# Autodesk Inventor assembly: Anglerfish_lunchbox_m12large_flipped_v0
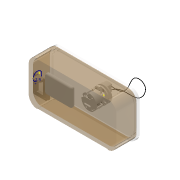
[picture p0: Inventor's stored thumbnail of the model, 180x180]
Saved by Autodesk Inventor 2022 (Build 260153000, 153)
## iProperties
Created: 2022-04-02
Part Number: Anglerfish_lunchbox_m12large_flipped_v0
Document SubType Name: Assembly
Designer: Prakash Lab
Author: Prakash Lab
## Documents named in this file (16)
- C:\Users\diederichbenedict\Dropbox\Dokumente\Promotion\PROJECTS\Matchboxscope\INVENTOR\RELEASE\Anglerfish\Workspace\Anglerfish_lunchbox_m12large_flipped_v0.iam
- C:\Users\diederichbenedict\Dropbox\Dokumente\Promotion\PROJECTS\Matchboxscope\INVENTOR\RELEASE\Anglerfish\Workspace\00_ESP3-CAM.iam
- C:\Users\diederichbenedict\Dropbox\Dokumente\Promotion\PROJECTS\Matchboxscope\INVENTOR\RELEASE\Anglerfish\Workspace\00_Powerbank.ipt
- C:\Users\diederichbenedict\Dropbox\Dokumente\Promotion\PROJECTS\Matchboxscope\INVENTOR\RELEASE\Anglerfish\Workspace\Matchboxscope_M12_Lensadapter_v0.ipt
- C:\Users\diederichbenedict\Dropbox\Dokumente\Promotion\PROJECTS\Matchboxscope\INVENTOR\RELEASE\Anglerfish\Workspace\00_CCTV_M12_VCM_large.ipt
- C:\Users\diederichbenedict\Dropbox\Dokumente\Promotion\PROJECTS\Matchboxscope\INVENTOR\RELEASE\Anglerfish\Workspace\Anglerfish_flipped_LidMoun.ipt
- C:\Users\diederichbenedict\Dropbox\Dokumente\Promotion\PROJECTS\Matchboxscope\INVENTOR\RELEASE\Anglerfish\Workspace\Anglerfish_flipped_Baselayer.ipt
- C:\Users\diederichbenedict\Dropbox\Dokumente\Promotion\PROJECTS\Matchboxscope\INVENTOR\RELEASE\Anglerfish\Workspace\Anglerfish_flipped_Electronicsmount.ipt
- C:\Users\diederichbenedict\Dropbox\Dokumente\Promotion\PROJECTS\Matchboxscope\INVENTOR\RELEASE\Anglerfish\Workspace\00_Magnet_8x3mm.ipt
- C:\Users\diederichbenedict\Dropbox\Dokumente\Promotion\PROJECTS\Matchboxscope\INVENTOR\RELEASE\Anglerfish\Workspace\DIN 912 - M3 x 0.5 x 12 x 10.75.ipt
- C:\Users\diederichbenedict\Dropbox\Dokumente\Promotion\PROJECTS\Matchboxscope\INVENTOR\RELEASE\Anglerfish\Workspace\00_Toslink.ipt
- C:\Users\diederichbenedict\Dropbox\Dokumente\Promotion\PROJECTS\Matchboxscope\INVENTOR\RELEASE\Anglerfish\Workspace\00_lunchbox_body.ipt
- C:\Users\diederichbenedict\Dropbox\Dokumente\Promotion\PROJECTS\Matchboxscope\INVENTOR\RELEASE\Anglerfish\Workspace\00_Lunchbox_cover.ipt
- C:\Users\diederichbenedict\Dropbox\Dokumente\Promotion\PROJECTS\Matchboxscope\INVENTOR\RELEASE\Anglerfish\Workspace\Matchboxscope_sample_universal_toslink.ipt
- C:\Users\diederichbenedict\Dropbox\Dokumente\Promotion\PROJECTS\Matchboxscope\INVENTOR\RELEASE\Anglerfish\Workspace\Anglerfish_coverslipclamp_top.ipt
- C:\Users\diederichbenedict\Dropbox\Dokumente\Promotion\PROJECTS\Matchboxscope\INVENTOR\RELEASE\Anglerfish\Workspace\Anglerfish_coverslipclamp_levelarm.ipt
## Components (27 placed, 15 different names)
1. 00_Powerbank:1
2. 00_ESP3-CAM:1 [sub-assembly] — Passend:23, Passend:24, Winkel:9, Winkel:11
3. 00_CCTV_M12_VCM_large:1 — Passend:30, Fluchtend:3, Einfügen:11
4. Matchboxscope_M12_Lensadapter_v0:1 — Einfügen:11
5. Anglerfish_flipped_Electronicsmount:1 — Einfügen:2, Winkel:11, Passend:30
6. Anglerfish_flipped_Baselayer:1 — Passend:23, Passend:24, Winkel:9, Einfügen:2, Winkel:10, Fluchtend:3, Einfügen:8, Einfügen:9, Einfügen:10, Einfügen:12, Einfügen:13, Einfügen:14, Einfügen:15, Einfügen:16, Einfügen:17, Einfügen:18
7. 00_Magnet_8x3mm:2 — Einfügen:21
8. 00_Magnet_8x3mm:3 — Einfügen:9
9. 00_Magnet_8x3mm:4 — Einfügen:20
10. 00_Magnet_8x3mm:5 — Einfügen:8
11. 00_Magnet_8x3mm:6 — Einfügen:10
12. DIN 912 - replaced by DIN EN ISO 4762 M3 x 12:1 — Einfügen:14
13. DIN 912 - replaced by DIN EN ISO 4762 M3 x 12:2 — Einfügen:17
14. DIN 912 - replaced by DIN EN ISO 4762 M3 x 12:4 — Einfügen:15
15. DIN 912 - replaced by DIN EN ISO 4762 M3 x 12:5 — Einfügen:12
16. DIN 912 - replaced by DIN EN ISO 4762 M3 x 12:6 — Einfügen:16
17. DIN 912 - replaced by DIN EN ISO 4762 M3 x 12:7 — Einfügen:13
18. 00_Toslink:1 — Einfügen:23
19. 00_lunchbox_body:1 — Fluchtend:4, Winkel:14, Fluchtend:33, Fluchtend:34, Passend:31
20. 00_Lunchbox_cover:1 — Fluchtend:33, Fluchtend:34, Passend:31, Fluchtend:35
21. Anglerfish_flipped_LidMoun:1 — Einfügen:18, Fluchtend:35, Einfügen:19, Einfügen:20, Einfügen:21, Einfügen:22
22. 00_Magnet_8x3mm:7 — Einfügen:19
23. Matchboxscope_M12_Lensadapter_v0:2 — Einfügen:24
24. Matchboxscope_sample_universal_toslink:2 — Einfügen:22, Einfügen:23, Einfügen:24
25. 00_Powerbank:2
26. Anglerfish_coverslipclamp_top:1 — Fluchtend:36, Fluchtend:37
27. Anglerfish_coverslipclamp_levelarm:1 — Fluchtend:36, Fluchtend:37
## Relationships (33: Insert 18, Flush 7, Mate 4, Angle 4)
- Passend:23 [Mate]: 00_ESP3-CAM:1 ↔ Anglerfish_flipped_Baselayer:1
- Passend:24 [Mate]: 00_ESP3-CAM:1 ↔ Anglerfish_flipped_Baselayer:1
- Winkel:9 [Angle] (180 deg): 00_ESP3-CAM:1 ↔ Anglerfish_flipped_Baselayer:1
- Einfügen:2 [Insert]: Anglerfish_flipped_Electronicsmount:1 ↔ Anglerfish_flipped_Baselayer:1
- Winkel:10 [Angle] (180 deg): Anglerfish_flipped_Baselayer:1
- Winkel:11 [Angle] (180 deg): 00_ESP3-CAM:1 ↔ Anglerfish_flipped_Electronicsmount:1
- Passend:30 [Mate]: 00_CCTV_M12_VCM_large:1 ↔ Anglerfish_flipped_Electronicsmount:1
- Fluchtend:3 [Flush]: 00_CCTV_M12_VCM_large:1 ↔ Anglerfish_flipped_Baselayer:1
- Einfügen:8 [Insert]: Anglerfish_flipped_Baselayer:1 ↔ 00_Magnet_8x3mm:5
- Einfügen:9 [Insert]: Anglerfish_flipped_Baselayer:1 ↔ 00_Magnet_8x3mm:3
- Einfügen:10 [Insert]: Anglerfish_flipped_Baselayer:1 ↔ 00_Magnet_8x3mm:6
- Einfügen:11 [Insert]: 00_CCTV_M12_VCM_large:1 ↔ Matchboxscope_M12_Lensadapter_v0:1
- Einfügen:12 [Insert]: Anglerfish_flipped_Baselayer:1 ↔ DIN 912 - replaced by DIN EN ISO 4762 M3 x 12:5
- Einfügen:13 [Insert]: Anglerfish_flipped_Baselayer:1 ↔ DIN 912 - replaced by DIN EN ISO 4762 M3 x 12:7
- Einfügen:14 [Insert]: Anglerfish_flipped_Baselayer:1 ↔ DIN 912 - replaced by DIN EN ISO 4762 M3 x 12:1
- Einfügen:15 [Insert]: Anglerfish_flipped_Baselayer:1 ↔ DIN 912 - replaced by DIN EN ISO 4762 M3 x 12:4
- Einfügen:16 [Insert]: Anglerfish_flipped_Baselayer:1 ↔ DIN 912 - replaced by DIN EN ISO 4762 M3 x 12:6
- Einfügen:17 [Insert]: Anglerfish_flipped_Baselayer:1 ↔ DIN 912 - replaced by DIN EN ISO 4762 M3 x 12:2
- Fluchtend:4 [Flush]: 00_lunchbox_body:1
- Winkel:14 [Angle] (180 deg): 00_lunchbox_body:1
- Fluchtend:33 [Flush]: 00_lunchbox_body:1 ↔ 00_Lunchbox_cover:1
- Fluchtend:34 [Flush]: 00_lunchbox_body:1 ↔ 00_Lunchbox_cover:1
- Passend:31 [Mate]: 00_lunchbox_body:1 ↔ 00_Lunchbox_cover:1
- Einfügen:18 [Insert] (-20 mm): Anglerfish_flipped_Baselayer:1 ↔ Anglerfish_flipped_LidMoun:1
- Fluchtend:35 [Flush] (-5 mm): 00_Lunchbox_cover:1 ↔ Anglerfish_flipped_LidMoun:1
- Einfügen:19 [Insert]: Anglerfish_flipped_LidMoun:1 ↔ 00_Magnet_8x3mm:7
- Einfügen:20 [Insert]: 00_Magnet_8x3mm:4 ↔ Anglerfish_flipped_LidMoun:1
- Einfügen:21 [Insert]: 00_Magnet_8x3mm:2 ↔ Anglerfish_flipped_LidMoun:1
- Einfügen:22 [Insert] (5 mm): Anglerfish_flipped_LidMoun:1 ↔ Matchboxscope_sample_universal_toslink:2
- Einfügen:23 [Insert]: 00_Toslink:1 ↔ Matchboxscope_sample_universal_toslink:2
- Einfügen:24 [Insert] (-20 mm): Matchboxscope_M12_Lensadapter_v0:2 ↔ Matchboxscope_sample_universal_toslink:2
- Fluchtend:36 [Flush]: Anglerfish_coverslipclamp_top:1 ↔ Anglerfish_coverslipclamp_levelarm:1
- Fluchtend:37 [Flush]: Anglerfish_coverslipclamp_top:1 ↔ Anglerfish_coverslipclamp_levelarm:1
